# Autodesk Inventor assembly: FrontWheelAssembly
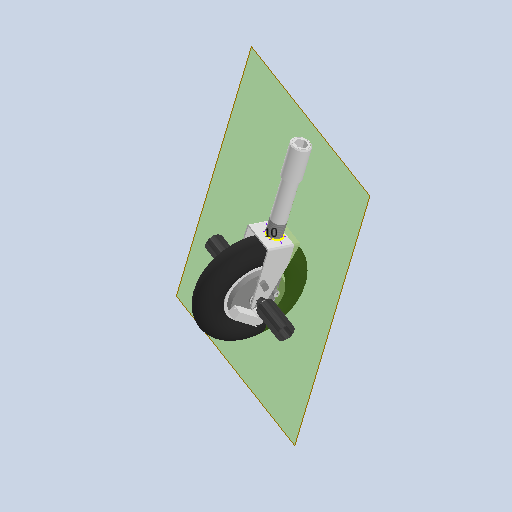
[picture p0: Inventor's stored thumbnail of the model, 512x512]
Saved by Autodesk Inventor 2022.2 (Build 262287000, 287)
## iProperties
Created: 2022-04-08
Part Number: FrontWheelAssembly
Document SubType Name: Assembly
Designer: Finn Oriwohl
Mass: 2612.45 g
Surface Area: 2901.63 cm^2
Volume: 1686.21 cm^3
Density: 1.5493 g/cm^3
Author: Finn Oriwohl
## Documents named in this file (4)
- H:\inventor ting\Mekatronik beercart git\Beercart CAD\Workspaces\Workspace\FrontWheelAssembly.iam
- H:\inventor ting\Mekatronik beercart git\Beercart CAD\Workspaces\Workspace\FreeBackWheel.ipt
- H:\inventor ting\Mekatronik beercart git\Beercart CAD\Workspaces\Workspace\pegsFront wheel.ipt
- H:\inventor ting\Mekatronik beercart git\Beercart CAD\Workspaces\Workspace\FrontWheelForkAssembly.iam
## Components (4 placed, 3 different names)
1. FreeBackWheel:1 — Insert:5
2. pegsFront wheel:1 — Insert:6
3. pegsFront wheel:2 — Insert:7
4. FrontWheelForkAssembly:1 [sub-assembly] — Insert:5, Insert:6, Insert:7, Angle:1, Tangent:1, Flush:1
## Relationships (6: Insert 3, Angle 1, Tangent 1, Flush 1)
- Insert:5: FreeBackWheel:1 ↔ FrontWheelForkAssembly:1
- Insert:6: pegsFront wheel:1 ↔ FrontWheelForkAssembly:1
- Insert:7: pegsFront wheel:2 ↔ FrontWheelForkAssembly:1
- Angle:1 (0 deg): FrontWheelForkAssembly:1
- Tangent:1: FrontWheelForkAssembly:1
- Flush:1: FrontWheelForkAssembly:1
